# Autodesk Inventor assembly: Omni Shaft
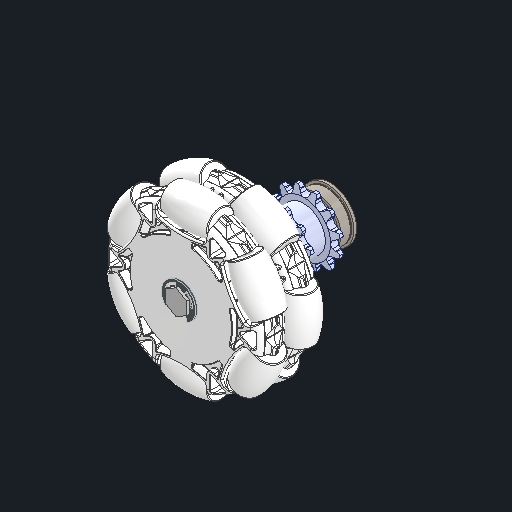
[picture p0: Inventor's stored thumbnail of the model, 512x512]
Saved by Autodesk Inventor 2022 (Build 260153000, 153)
## iProperties
Created: 2022-09-07
Part Number: Omni Shaft
Document SubType Name: Assembly
Designer: robpl
Author: robpl
## Documents named in this file (8)
- C:\Users\robpl\OneDrive\Documents\Inventor\WASP\Best Coast Drive\Omni Shaft.iam
- C:\Users\robpl\OneDrive\Documents\Inventor\WASP\Best Coast Drive\Omni Wheel Axle.ipt
- C:\Users\robpl\OneDrive\Documents\Inventor\WASP\Best Coast Drive\0.5 Flanged Hex Bearing (1.125 OD) (217-3875).ipt
- C:\Users\robpl\OneDrive\Documents\Inventor\WASP\Best Coast Drive\12T Steel Double Hub Sprocket (#35 Steel, 1_2_ Hex Bore) (217-5845) .ipt
- C:\Users\robpl\OneDrive\Documents\Inventor\WASP\Best Coast Drive\Omni Wheel\4_ Omni-Directional Wheel v2 (276-6194).iam
- C:\Users\robpl\OneDrive\Documents\Inventor\WASP\Best Coast Drive\3mm 0.5in Hex Spacer.ipt
- C:\Users\robpl\OneDrive\Documents\Inventor\WASP\Best Coast Drive\4.5mm 0.5in Hex Spacer.ipt
- C:\Users\robpl\OneDrive\Documents\Inventor\WASP\Best Coast Drive\10mm E-Clip.ipt
## Components (11 placed, 7 different names)
1. Omni Wheel Axle:1 — Mate:1, Mate:2, Flush:1, Mate:3, Mate:4, Mate:6, Mate:7, Flush:3, Mate:17, Mate:18, Mate:21, Mate:22, Mate:23, Mate:24, Flush:4
2. 0.5 Flanged Hex Bearing (1.125 OD) (217-3875):1 — Mate:3, Mate:4, Mate:10, Flush:3, Mate:13, Mate:14, Mate:16, Mate:20
3. 0.5 Flanged Hex Bearing (1.125 OD) (217-3875):2 — Mate:1, Mate:2, Flush:1, Mate:11, Mate:12
4. 12T Steel Double Hub Sprocket (#35 Steel, 1_2_ Hex Bore) (217-5845) :1 — Mate:6, Mate:7, Mate:10
5. 3mm 0.5in Hex Spacer:1 — Mate:11, Mate:12
6. 3mm 0.5in Hex Spacer:2 — Mate:13, Mate:14
7. 4.5mm 0.5in Hex Spacer:1 — Mate:16, Flush:4, Mate:25
8. 10mm E-Clip:1 — Mate:17, Mate:18
9. 10mm E-Clip:2 — Mate:19, Mate:22
10. 10mm E-Clip:3 — Mate:19, Mate:20, Mate:21
11. 4_ Omni-Directional Wheel v2 (276-6194):1 [sub-assembly] — Mate:23, Mate:24, Mate:25
## Relationships (24: Mate 21, Flush 3)
- Mate:1: Omni Wheel Axle:1 ↔ 0.5 Flanged Hex Bearing (1.125 OD) (217-3875):2
- Mate:2: Omni Wheel Axle:1 ↔ 0.5 Flanged Hex Bearing (1.125 OD) (217-3875):2
- Flush:1: Omni Wheel Axle:1 ↔ 0.5 Flanged Hex Bearing (1.125 OD) (217-3875):2
- Mate:3: Omni Wheel Axle:1 ↔ 0.5 Flanged Hex Bearing (1.125 OD) (217-3875):1
- Mate:4: Omni Wheel Axle:1 ↔ 0.5 Flanged Hex Bearing (1.125 OD) (217-3875):1
- Mate:6: Omni Wheel Axle:1 ↔ 12T Steel Double Hub Sprocket (#35 Steel, 1_2_ Hex Bore) (217-5845) :1
- Mate:7: Omni Wheel Axle:1 ↔ 12T Steel Double Hub Sprocket (#35 Steel, 1_2_ Hex Bore) (217-5845) :1
- Mate:10 (3 mm): 0.5 Flanged Hex Bearing (1.125 OD) (217-3875):1 ↔ 12T Steel Double Hub Sprocket (#35 Steel, 1_2_ Hex Bore) (217-5845) :1
- Flush:3: Omni Wheel Axle:1 ↔ 0.5 Flanged Hex Bearing (1.125 OD) (217-3875):1
- Mate:11: 0.5 Flanged Hex Bearing (1.125 OD) (217-3875):2 ↔ 3mm 0.5in Hex Spacer:1
- Mate:12: 0.5 Flanged Hex Bearing (1.125 OD) (217-3875):2 ↔ 3mm 0.5in Hex Spacer:1
- Mate:13: 0.5 Flanged Hex Bearing (1.125 OD) (217-3875):1 ↔ 3mm 0.5in Hex Spacer:2
- Mate:14: 0.5 Flanged Hex Bearing (1.125 OD) (217-3875):1 ↔ 3mm 0.5in Hex Spacer:2
- Mate:16: 0.5 Flanged Hex Bearing (1.125 OD) (217-3875):1 ↔ 4.5mm 0.5in Hex Spacer:1
- Mate:17: Omni Wheel Axle:1 ↔ 10mm E-Clip:1
- Mate:18: Omni Wheel Axle:1 ↔ 10mm E-Clip:1
- Mate:19: 10mm E-Clip:2 ↔ 10mm E-Clip:3
- Mate:20: 0.5 Flanged Hex Bearing (1.125 OD) (217-3875):1 ↔ 10mm E-Clip:3
- Mate:21: Omni Wheel Axle:1 ↔ 10mm E-Clip:3
- Mate:22: Omni Wheel Axle:1 ↔ 10mm E-Clip:2
- Mate:23: Omni Wheel Axle:1 ↔ 4_ Omni-Directional Wheel v2 (276-6194):1
- Mate:24: Omni Wheel Axle:1 ↔ 4_ Omni-Directional Wheel v2 (276-6194):1
- Flush:4: Omni Wheel Axle:1 ↔ 4.5mm 0.5in Hex Spacer:1
- Mate:25: 4.5mm 0.5in Hex Spacer:1 ↔ 4_ Omni-Directional Wheel v2 (276-6194):1
